# Autodesk Inventor assembly: parallel manipulator
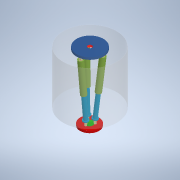
[picture p0: Inventor's stored thumbnail of the model, 180x180]
Saved by Autodesk Inventor 2020 (Build 240168000, 168)
## iProperties
Created: 2020-12-11
Part Number: parallel manipulator
Document SubType Name: Assembly
Designer: Vikki
Author: Vikki
## Documents named in this file (9)
- E:\borewell rescuebot\pll manipulator files\sps manipulator\parallel manipulator.iam
- E:\borewell rescuebot\pll manipulator files\sps manipulator\well.ipt
- E:\borewell rescuebot\pll manipulator files\sps manipulator\well maximum size.ipt
- E:\borewell rescuebot\pll manipulator files\sps manipulator\pll-base.ipt
- E:\borewell rescuebot\pll manipulator files\sps manipulator\pll-end eff.ipt
- E:\borewell rescuebot\pll manipulator files\sps manipulator\borewell max size.ipt
- E:\borewell rescuebot\pll manipulator files\sps manipulator\pin.ipt
- E:\borewell rescuebot\pll manipulator files\sps manipulator\piston v1.ipt
- E:\borewell rescuebot\pll manipulator files\sps manipulator\plunger v1.ipt
## Components (12 placed, 8 different names)
1. well:1 — Flush:1, Mate:10
2. well maximum size:1 — Flush:1, Flush:2, Mate:2
3. pll-base:1 — Flush:2, Mate:2, Angle:1, Mate:9, Mate:12, Flush:3, Angle:3, Mate:14, Mate:17, Mate:18
4. pll-end eff:1 — Angle:1, Mate:9, Mate:10, Mate:11, Angle:3, Mate:20, Mate:21, Mate:22, Mate:23
5. pin:1 — Mate:11
6. borewell max size:1 — Mate:12, Flush:3
7. piston v1:1 — Mate:14
8. plunger v1:1 — Mate:23
9. piston v1:2 — Mate:17
10. plunger v1:2 — Mate:20, Mate:21
11. piston v1:3 — Mate:18
12. plunger v1:3 — Mate:22
## Relationships (20: Mate 15, Flush 3, Angle 2)
- Flush:1: well:1 ↔ well maximum size:1
- Flush:2: well maximum size:1 ↔ pll-base:1
- Mate:2: well maximum size:1 ↔ pll-base:1
- Angle:1 (180 deg): pll-base:1 ↔ pll-end eff:1
- Mate:9: pll-base:1 ↔ pll-end eff:1
- Mate:10: well:1 ↔ pll-end eff:1
- Mate:11: pll-end eff:1 ↔ pin:1
- Mate:12: pll-base:1 ↔ borewell max size:1
- Flush:3: pll-base:1 ↔ borewell max size:1
- Angle:3 (0 deg): pll-base:1 ↔ pll-end eff:1
- [Mate]: piston v1:1 ↔ plunger v1:1
- Mate:14: pll-base:1 ↔ piston v1:1
- [Mate]: piston v1:2 ↔ plunger v1:2
- [Mate]: piston v1:3 ↔ plunger v1:3
- Mate:17: pll-base:1 ↔ piston v1:2
- Mate:18: pll-base:1 ↔ piston v1:3
- Mate:20: pll-end eff:1 ↔ plunger v1:2
- Mate:21: pll-end eff:1 ↔ plunger v1:2
- Mate:22: pll-end eff:1 ↔ plunger v1:3
- Mate:23: pll-end eff:1 ↔ plunger v1:1
## Named parameters: d27_d1 = 0 mm, d29_d1 = 0 mm, d30_d1 = 0 mm
